# Autodesk Inventor assembly: fourbardraft_MIR_MIR
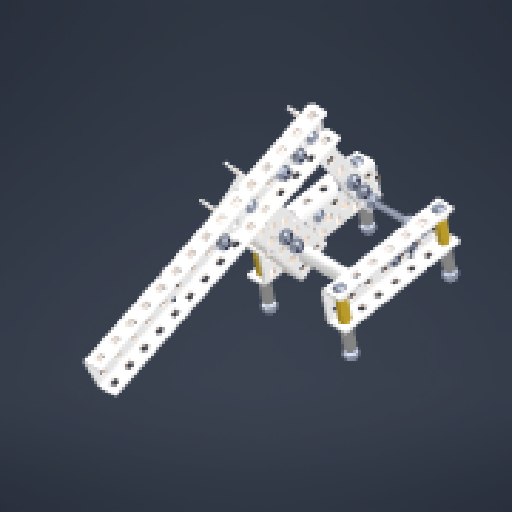
[picture p0: Inventor's stored thumbnail of the model, 512x512]
Saved by Autodesk Inventor 2023 (Build 270158000, 158)
## iProperties
Created: 2023-08-09
Part Number: fourbardraft_MIR_MIR
Document SubType Name: Assembly
Designer: srbel
Author: srbel
## Documents named in this file (18)
- C:\CAD\OverUnderCAD\Drive\fourbardraft_MIR_MIR.iam
- C:\CAD\OverUnderCAD\VEX-CAD-Inventor-1.4.0\Structure\C Channel\Aluminum 1x2x1\Alu C 1x2x1x6_MIR2_MIR.ipt
- C:\CAD\OverUnderCAD\Drive\fourbarintakebearing_MIR2_MIR1_MIR_MIR.iam
- C:\CAD\OverUnderCAD\Drive\fourbarintakebearing_MIR_MIR1_MIR1_MIR_MIR.iam
- C:\CAD\OverUnderCAD\VEX-CAD-Inventor-1.4.0\Motion\Shaft LS\Bearing Flat_MIR5_MIR1_MIR_MIR.ipt
- C:\CAD\OverUnderCAD\VEX-CAD-Inventor-1.4.0\Structure\C Channel\Aluminum 1x2x1\Alu C 1x2x1x8_MIR2_MIR1_MIR_MIR.ipt
- C:\CAD\OverUnderCAD\VEX-CAD-Inventor-1.4.0\Motion\Spacers\Spacer Nylon .313 OD\NSpacer .313 OD x .250.ipt
- C:\CAD\OverUnderCAD\VEX-CAD-Inventor-1.4.0\Motion\Spacers\Spacer Nylon .313 OD.ipt
- C:\CAD\OverUnderCAD\VEX-CAD-Inventor-1.4.0\Structure\Angle\Aluminum\1x1\Alu Angle 1x1x8_MIR2_MIR1_MIR_MIR.ipt
- C:\CAD\OverUnderCAD\VEX-CAD-Inventor-1.4.0\Structure\C Channel\Aluminum 1x2x1\Alu C 1x2x1x15_MIR1_MIR1_MIR_MIR.ipt
- C:\CAD\OverUnderCAD\VEX-CAD-Inventor-1.4.0\Motion\Shaft LS\Bearing Flat_MIR3_MIR1_MIR1_MIR_MIR.ipt
- C:\CAD\OverUnderCAD\VEX-CAD-Inventor-1.4.0\Structure\Hardware\Nut Thin Nylock_MIR7_MIR1_MIR1_MIR_MIR1.ipt
- C:\CAD\OverUnderCAD\VEX-CAD-Inventor-1.4.0\Structure\Hardware\Screw Steel - Star\SScrew Star Threaded .500.ipt
- C:\CAD\OverUnderCAD\VEX-CAD-Inventor-1.4.0\Structure\Hardware\Screw Steel - Star.ipt
- C:\CAD\OverUnderCAD\VEX-CAD-Inventor-1.4.0\Motion\Spacers\Washer Teflon\TWasher .375 OD x .06250.ipt
- C:\CAD\OverUnderCAD\VEX-CAD-Inventor-1.4.0\Motion\Spacers\Washer Teflon.ipt
- C:\CAD\OverUnderCAD\VEX-CAD-Inventor-1.4.0\Structure\Hardware\Screw Steel - Star\SScrew Star Threaded 2.500.ipt
- C:\CAD\OverUnderCAD\VEX-CAD-Inventor-1.4.0\Motion\Spacers\Spacer Nylon .313 OD\NSpacer .313 OD x .500.ipt
## Components (46 placed, 14 different names)
1. Alu C 1x2x1x6_MIR2_MIR:1
2. fourbarintakebearing_MIR2_MIR1_MIR_MIR:1 [sub-assembly] — Insert:173, Insert:199, Insert:201, Insert:54
3. fourbarintakebearing_MIR_MIR1_MIR1_MIR_MIR:1 [sub-assembly] — Insert:183, Insert:185, Insert:186, Insert:196, Insert:219, Insert:59
4. Bearing Flat_MIR5_MIR1_MIR_MIR:1 — Insert:170, Insert:171, Insert:172, Insert:192, Insert:193
5. Alu C 1x2x1x8_MIR2_MIR1_MIR_MIR:1 — Insert:170, Insert:171, Insert:178, Insert:194, Insert:195, Insert:217
6. NSpacer .313 OD x .250:1 — Insert:172, Insert:173
7. Bearing Flat_MIR5_MIR1_MIR_MIR:2 — Insert:174, Insert:175, Insert:189, Insert:190, Insert:53
8. Alu Angle 1x1x8_MIR2_MIR1_MIR_MIR:1 — Insert:174, Insert:175, Insert:55, Insert:188, Insert:191, Insert:57, Insert:58
9. Alu C 1x2x1x15_MIR1_MIR1_MIR_MIR:1 — Insert:55, Insert:178, Insert:179, Insert:180, Insert:207, Insert:209, Insert:212, Insert:214, Insert:215
10. Bearing Flat_MIR5_MIR1_MIR_MIR:3 — Insert:179, Insert:180, Insert:208, Insert:210, Insert:56
11. Bearing Flat_MIR3_MIR1_MIR1_MIR_MIR:1 — Insert:183, Insert:184, Insert:187, Insert:200
12. Nut Thin Nylock_MIR7_MIR1_MIR1_MIR_MIR1:1 — Insert:184
13. SScrew Star Threaded .500:1 — Insert:185
14. SScrew Star Threaded .500:2 — Insert:186
15. Nut Thin Nylock_MIR7_MIR1_MIR1_MIR_MIR1:2 — Insert:187
16. Nut Thin Nylock_MIR7_MIR1_MIR1_MIR_MIR1:3 — Insert:188
17. SScrew Star Threaded .500:3 — Insert:189
18. SScrew Star Threaded .500:4 — Insert:190
19. Nut Thin Nylock_MIR7_MIR1_MIR1_MIR_MIR1:4 — Insert:191
20. SScrew Star Threaded .500:5 — Insert:192
21. SScrew Star Threaded .500:6 — Insert:193
22. Nut Thin Nylock_MIR7_MIR1_MIR1_MIR_MIR1:5 — Insert:194
23. Nut Thin Nylock_MIR7_MIR1_MIR1_MIR_MIR1:6 — Insert:195
24. Nut Thin Nylock_MIR7_MIR1_MIR1_MIR_MIR1:7 — Insert:197
25. TWasher .375 OD x .06250:1 — Insert:196, Insert:197
26. Nut Thin Nylock_MIR7_MIR1_MIR1_MIR_MIR1:8 — Insert:198
27. TWasher .375 OD x .06250:2 — Insert:198, Insert:199
28. SScrew Star Threaded 2.500:7 — Insert:200
29. SScrew Star Threaded 2.500:8 — Insert:201
30. SScrew Star Threaded .500:9 — Insert:207
31. Nut Thin Nylock_MIR7_MIR1_MIR1_MIR_MIR1:9 — Insert:208
32. SScrew Star Threaded .500:10 — Insert:209
33. Nut Thin Nylock_MIR7_MIR1_MIR1_MIR_MIR1:10 — Insert:210
34. SScrew Star Threaded .500:11 — Insert:211, Insert:216
35. Nut Thin Nylock_MIR7_MIR1_MIR1_MIR_MIR1:11 — Insert:211
36. SScrew Star Threaded .500:12 — Insert:212, Insert:213
37. Nut Thin Nylock_MIR7_MIR1_MIR1_MIR_MIR1:12 — Insert:213
38. Bearing Flat_MIR5_MIR1_MIR_MIR:4 — Insert:214, Insert:215, Insert:216
39. NSpacer .313 OD x .500:2 — Insert:217, Insert:218
40. NSpacer .313 OD x .250:3 — Insert:218, Insert:220
41. NSpacer .313 OD x .500:4 — Insert:219, Insert:220
42. NSpacer .313 OD x .250:5 — Insert:54, Insert:53
43. Nut Thin Nylock_MIR7_MIR1_MIR1_MIR_MIR1:13 — Insert:57
44. SScrew Star Threaded .500:13 — Insert:56
45. Nut Thin Nylock_MIR7_MIR1_MIR1_MIR_MIR1:14 — Insert:58
46. Nut Thin Nylock_MIR7_MIR1_MIR1_MIR_MIR1:15 — Insert:59
## Relationships (49: Insert 49)
- Insert:170: Bearing Flat_MIR5_MIR1_MIR_MIR:1 ↔ Alu C 1x2x1x8_MIR2_MIR1_MIR_MIR:1
- Insert:171: Bearing Flat_MIR5_MIR1_MIR_MIR:1 ↔ Alu C 1x2x1x8_MIR2_MIR1_MIR_MIR:1
- Insert:172: Bearing Flat_MIR5_MIR1_MIR_MIR:1 ↔ NSpacer .313 OD x .250:1
- Insert:173: fourbarintakebearing_MIR2_MIR1_MIR_MIR:1 ↔ NSpacer .313 OD x .250:1
- Insert:174: Bearing Flat_MIR5_MIR1_MIR_MIR:2 ↔ Alu Angle 1x1x8_MIR2_MIR1_MIR_MIR:1
- Insert:175: Bearing Flat_MIR5_MIR1_MIR_MIR:2 ↔ Alu Angle 1x1x8_MIR2_MIR1_MIR_MIR:1
- Insert:55: Alu Angle 1x1x8_MIR2_MIR1_MIR_MIR:1 ↔ Alu C 1x2x1x15_MIR1_MIR1_MIR_MIR:1
- Insert:178: Alu C 1x2x1x8_MIR2_MIR1_MIR_MIR:1 ↔ Alu C 1x2x1x15_MIR1_MIR1_MIR_MIR:1
- Insert:179: Alu C 1x2x1x15_MIR1_MIR1_MIR_MIR:1 ↔ Bearing Flat_MIR5_MIR1_MIR_MIR:3
- Insert:180: Alu C 1x2x1x15_MIR1_MIR1_MIR_MIR:1 ↔ Bearing Flat_MIR5_MIR1_MIR_MIR:3
- Insert:183: fourbarintakebearing_MIR_MIR1_MIR1_MIR_MIR:1 ↔ Bearing Flat_MIR3_MIR1_MIR1_MIR_MIR:1
- Insert:184: Bearing Flat_MIR3_MIR1_MIR1_MIR_MIR:1 ↔ Nut Thin Nylock_MIR7_MIR1_MIR1_MIR_MIR1:1
- Insert:185: fourbarintakebearing_MIR_MIR1_MIR1_MIR_MIR:1 ↔ SScrew Star Threaded .500:1
- Insert:186: fourbarintakebearing_MIR_MIR1_MIR1_MIR_MIR:1 ↔ SScrew Star Threaded .500:2
- Insert:187: Bearing Flat_MIR3_MIR1_MIR1_MIR_MIR:1 ↔ Nut Thin Nylock_MIR7_MIR1_MIR1_MIR_MIR1:2
- Insert:188: Alu Angle 1x1x8_MIR2_MIR1_MIR_MIR:1 ↔ Nut Thin Nylock_MIR7_MIR1_MIR1_MIR_MIR1:3
- Insert:189: Bearing Flat_MIR5_MIR1_MIR_MIR:2 ↔ SScrew Star Threaded .500:3
- Insert:190: Bearing Flat_MIR5_MIR1_MIR_MIR:2 ↔ SScrew Star Threaded .500:4
- Insert:191: Alu Angle 1x1x8_MIR2_MIR1_MIR_MIR:1 ↔ Nut Thin Nylock_MIR7_MIR1_MIR1_MIR_MIR1:4
- Insert:192: Bearing Flat_MIR5_MIR1_MIR_MIR:1 ↔ SScrew Star Threaded .500:5
- Insert:193: Bearing Flat_MIR5_MIR1_MIR_MIR:1 ↔ SScrew Star Threaded .500:6
- Insert:194: Alu C 1x2x1x8_MIR2_MIR1_MIR_MIR:1 ↔ Nut Thin Nylock_MIR7_MIR1_MIR1_MIR_MIR1:5
- Insert:195: Alu C 1x2x1x8_MIR2_MIR1_MIR_MIR:1 ↔ Nut Thin Nylock_MIR7_MIR1_MIR1_MIR_MIR1:6
- Insert:196: fourbarintakebearing_MIR_MIR1_MIR1_MIR_MIR:1 ↔ TWasher .375 OD x .06250:1
- Insert:197: Nut Thin Nylock_MIR7_MIR1_MIR1_MIR_MIR1:7 ↔ TWasher .375 OD x .06250:1
- Insert:198: Nut Thin Nylock_MIR7_MIR1_MIR1_MIR_MIR1:8 ↔ TWasher .375 OD x .06250:2
- Insert:199: fourbarintakebearing_MIR2_MIR1_MIR_MIR:1 ↔ TWasher .375 OD x .06250:2
- Insert:200: Bearing Flat_MIR3_MIR1_MIR1_MIR_MIR:1 ↔ SScrew Star Threaded 2.500:7
- Insert:201: fourbarintakebearing_MIR2_MIR1_MIR_MIR:1 ↔ SScrew Star Threaded 2.500:8
- Insert:207: Alu C 1x2x1x15_MIR1_MIR1_MIR_MIR:1 ↔ SScrew Star Threaded .500:9
- Insert:208: Bearing Flat_MIR5_MIR1_MIR_MIR:3 ↔ Nut Thin Nylock_MIR7_MIR1_MIR1_MIR_MIR1:9
- Insert:209: Alu C 1x2x1x15_MIR1_MIR1_MIR_MIR:1 ↔ SScrew Star Threaded .500:10
- Insert:210: Bearing Flat_MIR5_MIR1_MIR_MIR:3 ↔ Nut Thin Nylock_MIR7_MIR1_MIR1_MIR_MIR1:10
- Insert:211 (8.3185 mm): SScrew Star Threaded .500:11 ↔ Nut Thin Nylock_MIR7_MIR1_MIR1_MIR_MIR1:11
- Insert:212: Alu C 1x2x1x15_MIR1_MIR1_MIR_MIR:1 ↔ SScrew Star Threaded .500:12
- Insert:213 (8.3185 mm): SScrew Star Threaded .500:12 ↔ Nut Thin Nylock_MIR7_MIR1_MIR1_MIR_MIR1:12
- Insert:214: Alu C 1x2x1x15_MIR1_MIR1_MIR_MIR:1 ↔ Bearing Flat_MIR5_MIR1_MIR_MIR:4
- Insert:215: Alu C 1x2x1x15_MIR1_MIR1_MIR_MIR:1 ↔ Bearing Flat_MIR5_MIR1_MIR_MIR:4
- Insert:216: SScrew Star Threaded .500:11 ↔ Bearing Flat_MIR5_MIR1_MIR_MIR:4
- Insert:217: Alu C 1x2x1x8_MIR2_MIR1_MIR_MIR:1 ↔ NSpacer .313 OD x .500:2
- Insert:218: NSpacer .313 OD x .500:2 ↔ NSpacer .313 OD x .250:3
- Insert:219: fourbarintakebearing_MIR_MIR1_MIR1_MIR_MIR:1 ↔ NSpacer .313 OD x .500:4
- Insert:220: NSpacer .313 OD x .250:3 ↔ NSpacer .313 OD x .500:4
- Insert:54: fourbarintakebearing_MIR2_MIR1_MIR_MIR:1 ↔ NSpacer .313 OD x .250:5
- Insert:53: Bearing Flat_MIR5_MIR1_MIR_MIR:2 ↔ NSpacer .313 OD x .250:5
- Insert:57: Alu Angle 1x1x8_MIR2_MIR1_MIR_MIR:1 ↔ Nut Thin Nylock_MIR7_MIR1_MIR1_MIR_MIR1:13
- Insert:56: Bearing Flat_MIR5_MIR1_MIR_MIR:3 ↔ SScrew Star Threaded .500:13
- Insert:58: Alu Angle 1x1x8_MIR2_MIR1_MIR_MIR:1 ↔ Nut Thin Nylock_MIR7_MIR1_MIR1_MIR_MIR1:14
- Insert:59: fourbarintakebearing_MIR_MIR1_MIR1_MIR_MIR:1 ↔ Nut Thin Nylock_MIR7_MIR1_MIR1_MIR_MIR1:15
